# Autodesk Inventor assembly: Module PCB with keepout
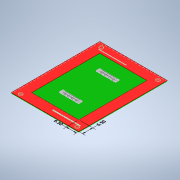
[picture p0: Inventor's stored thumbnail of the model, 180x180]
Saved by Autodesk Inventor 2022 (Build 260153000, 153)
## iProperties
Created: 2022-02-26
Part Number: Module PCB with keepout
Document SubType Name: Assembly
Designer: Caleb
Author: Caleb
## Documents named in this file (3)
- C:\Users\Caleb\Desktop\nebraska-silicon-lab\Hardware\ETL\modules\tamale\Module PCB with keepout.iam
- C:\Users\Caleb\Desktop\nebraska-silicon-lab\Hardware\ETL\modules\tamale\Mock Module PCB - V2p1.iam
- C:\Users\Caleb\Desktop\nebraska-silicon-lab\Hardware\ETL\modules\tamale\smt_keepout.ipt
## Components (2 placed, 2 different names)
1. Mock Module PCB - V2p1:1 [sub-assembly] — Mate:1, Flush:1, Flush:2
2. smt_keepout:1 — Mate:1, Flush:1, Flush:2
## Relationships (3: Flush 2, Mate 1)
- Mate:1: Mock Module PCB - V2p1:1 ↔ smt_keepout:1
- Flush:1: Mock Module PCB - V2p1:1 ↔ smt_keepout:1
- Flush:2: Mock Module PCB - V2p1:1 ↔ smt_keepout:1
